# Autodesk Inventor assembly: Ensamble lab DInámica
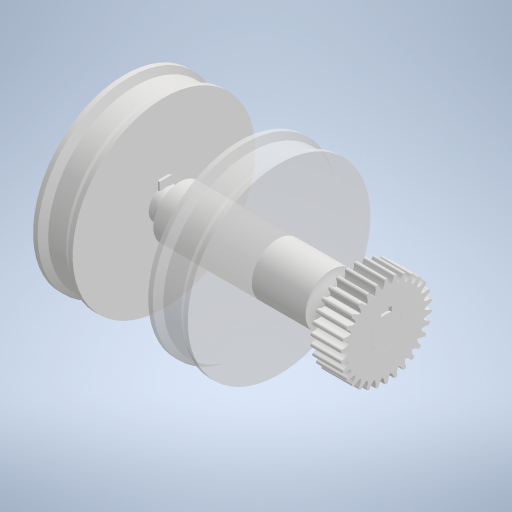
[picture p0: Inventor's stored thumbnail of the model, 512x512]
Saved by Autodesk Inventor 2024.2 (Build 282272000, 272)
## iProperties
Created: 2024-03-27
Part Number: Ensamble lab DInámica
Document SubType Name: Assembly
Designer: ashju
Author: ashju
## Documents named in this file (6)
- C:\Users\ashju\OneDrive\Documentos\Ensamble lab DInámica.iam
- C:\Users\ashju\Downloads\POLEA (1).ipt
- C:\Users\ashju\Downloads\ENGRANE (1).ipt
- C:\Users\ashju\Downloads\CUÑA (1).ipt
- C:\Users\ashju\Downloads\EJE_CUÑEROS (1).ipt
- C:\Users\ashju\OneDrive\Documentos\ensamble 1\Design Accelerator\Worm Gears1.iam
## Components (7 placed, 5 different names)
1. POLEA (1):1 — Rotational:1
2. CUÑA (1):1 — Rigid:1
3. EJE_CUÑEROS (1):1 — Rotational:1, Rotational:2, Rigid:1, Rigid:2
4. CUÑA (1):2 — Rigid:2
5. Worm Gears:1 [sub-assembly]
6. POLEA (1):2
7. ENGRANE (1):1 — Rotational:2
## Relationships (4: RevoluteJoint 2, WeldJoint 2)
- Rotational:1 [RevoluteJoint]: POLEA (1):1 ↔ EJE_CUÑEROS (1):1
- Rotational:2 [RevoluteJoint]: EJE_CUÑEROS (1):1 ↔ ENGRANE (1):1
- Rigid:1 [WeldJoint]: CUÑA (1):1 ↔ EJE_CUÑEROS (1):1
- Rigid:2 [WeldJoint]: EJE_CUÑEROS (1):1 ↔ CUÑA (1):2
